# Autodesk Inventor assembly: tire_out
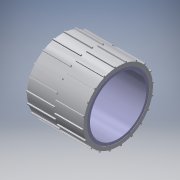
[picture p0: Inventor's stored thumbnail of the model, 180x180]
Saved by Autodesk Inventor 2018 (Build 220112000, 112)
## iProperties
Created: 2017-09-12
Part Number: tire_out
Material: 一般
Document SubType Name: Assembly
Designer: 翔
Source: UnKnown
Author: 翔
## Documents named in this file (4)
- E:\forest_robot_cad\Forest_v4\wheel\tire_out.iam
- E:\forest_robot_cad\terzo tentativo\plate_wheel.ipt
- E:\forest_robot_cad\Forest_v4\wheel\Wheel.ipt
- E:\forest_robot_cad\Forest_v4\wheel\tire.ipt
## Components (3 placed, 3 different names)
1. plate_wheel.1 — メイト:1, メイト:2, フラッシュ:1, フラッシュ:2
2. Part1.1 — メイト:1, メイト:2, フラッシュ:1, メイト:3
3. tire.1 — メイト:3, フラッシュ:2
## Relationships (5: Mate 3, Flush 2)
- メイト:1 [Mate]: plate_wheel.1 ↔ Part1.1
- メイト:2 [Mate]: plate_wheel.1 ↔ Part1.1
- フラッシュ:1 [Flush]: plate_wheel.1 ↔ Part1.1
- メイト:3 [Mate]: Part1.1 ↔ tire.1
- フラッシュ:2 [Flush]: plate_wheel.1 ↔ tire.1
